# Autodesk Inventor assembly: ExtendedBracket
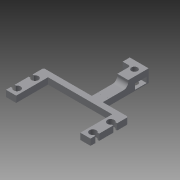
[picture p0: Inventor's stored thumbnail of the model, 180x180]
Saved by Autodesk Inventor 2014 SP1 (Build 180222100, 222)
## iProperties
Created: 2017-02-23
Part Number: ExtendedBracket
Document SubType Name: Assembly
Designer: danielsikar
Author: danielsikar
## Documents named in this file (3)
- C:\Users\danielsikar\Documents\Projects\iot-graffiti\cad\assemblies\ExtendedBracket.iam
- C:\Users\danielsikar\Documents\Projects\iot-graffiti\cad\parts\MG996RBracketTop.ipt
- C:\Users\danielsikar\Documents\Projects\iot-graffiti\cad\parts\MG996RBracketBottom.ipt
## Components (2 placed, 2 different names)
1. MG996RBracketTop:1 — Mate:1, Mate:2, Mate:3, Flush:1, Mate:5
2. MG996RBracketBottom:1 — Mate:4, Flush:1, Mate:5
## Relationships (6: Mate 5, Flush 1)
- Mate:1: MG996RBracketTop:1
- Mate:2: MG996RBracketTop:1
- Mate:3: MG996RBracketTop:1
- Mate:4: MG996RBracketBottom:1
- Flush:1: MG996RBracketTop:1 ↔ MG996RBracketBottom:1
- Mate:5 (3.4 mm): MG996RBracketTop:1 ↔ MG996RBracketBottom:1
